# Autodesk Inventor assembly: Pull Tester
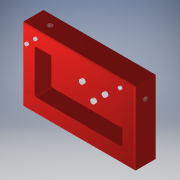
[picture p0: Inventor's stored thumbnail of the model, 180x180]
Saved by Autodesk Inventor 2019.4 (Build 234330000, 330)
## iProperties
Created: 2020-11-12
Part Number: Pull Tester
Document SubType Name: Assembly
Designer: caleb
Author: caleb
## Documents named in this file (5)
- C:\Users\cfang\Desktop\nebraska-silicon-lab\CAD\Pull Tester\Pull Tester.iam
- C:\Users\cfang\Desktop\nebraska-silicon-lab\CAD\Pull Tester\Chuck.ipt
- C:\Users\cfang\Desktop\nebraska-silicon-lab\CAD\Pull Tester\step_12692.ipt
- C:\Users\cfang\Desktop\nebraska-silicon-lab\CAD\Pull Tester\90128A263_ZNC-PLTD ALLOY STL SCKT HEAD CAP SCREW.ipt
- C:\Users\cfang\Desktop\nebraska-silicon-lab\CAD\Pull Tester\90128A211_ZNC-PLTD ALLOY STL SCKT HEAD CAP SCREW.ipt
## Components (9 placed, 4 different names)
1. Chuck:1 — Mate:1, Angle:1, Insert:17, Insert:18, Insert:19, Insert:20, Insert:21, Insert:22, Insert:23, Insert:24
2. step_12692:1 — Mate:1, Angle:1, Insert:17
3. 90128A263_ZNC-PLTD ALLOY STL SCKT HEAD CAP SCREW:1 — Insert:18
4. 90128A263_ZNC-PLTD ALLOY STL SCKT HEAD CAP SCREW:2 — Insert:21
5. 90128A263_ZNC-PLTD ALLOY STL SCKT HEAD CAP SCREW:3 — Insert:20
6. 90128A263_ZNC-PLTD ALLOY STL SCKT HEAD CAP SCREW:4 — Insert:19
7. 90128A211_ZNC-PLTD ALLOY STL SCKT HEAD CAP SCREW:1 — Insert:24
8. 90128A211_ZNC-PLTD ALLOY STL SCKT HEAD CAP SCREW:2 — Insert:23
9. 90128A211_ZNC-PLTD ALLOY STL SCKT HEAD CAP SCREW:3 — Insert:22
## Relationships (10: Insert 8, Mate 1, Angle 1)
- Mate:1: Chuck:1 ↔ step_12692:1
- Angle:1 (0 deg): Chuck:1 ↔ step_12692:1
- Insert:17: Chuck:1 ↔ step_12692:1
- Insert:18: Chuck:1 ↔ 90128A263_ZNC-PLTD ALLOY STL SCKT HEAD CAP SCREW:1
- Insert:19: Chuck:1 ↔ 90128A263_ZNC-PLTD ALLOY STL SCKT HEAD CAP SCREW:4
- Insert:20: Chuck:1 ↔ 90128A263_ZNC-PLTD ALLOY STL SCKT HEAD CAP SCREW:3
- Insert:21: Chuck:1 ↔ 90128A263_ZNC-PLTD ALLOY STL SCKT HEAD CAP SCREW:2
- Insert:22: Chuck:1 ↔ 90128A211_ZNC-PLTD ALLOY STL SCKT HEAD CAP SCREW:3
- Insert:23: Chuck:1 ↔ 90128A211_ZNC-PLTD ALLOY STL SCKT HEAD CAP SCREW:2
- Insert:24: Chuck:1 ↔ 90128A211_ZNC-PLTD ALLOY STL SCKT HEAD CAP SCREW:1
